# Autodesk Inventor assembly: solenoid
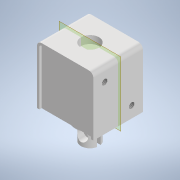
[picture p0: Inventor's stored thumbnail of the model, 180x180]
Saved by Autodesk Inventor 2021 (Build 250183000, 183)
## iProperties
Created: 2020-06-26
Part Number: solenoid
Document SubType Name: Assembly
Designer: Yatekii
Author: Yatekii
## Documents named in this file (3)
- C:\Users\Yatekii\repos\rcache\solenoid\solenoid.iam
- C:\Users\Yatekii\repos\rcache\solenoid\main_block.ipt
- C:\Users\Yatekii\repos\rcache\solenoid\pole.ipt
## Components (2 placed, 2 different names)
1. main_block:1 — Cylindrical:1
2. pole:1 — Cylindrical:1
## Relationships (1: CylindricalJoint 1)
- Cylindrical:1: main_block:1 ↔ pole:1
